# Autodesk Inventor assembly: X_CarriageR_V2_0
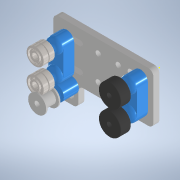
[picture p0: Inventor's stored thumbnail of the model, 180x180]
Saved by Autodesk Inventor 2021 (Build 250183000, 183)
## iProperties
Created: 2021-06-13
Part Number: X_CarriageR_V2_0
Document SubType Name: Assembly
Designer: Jorian Brusind
Author: Jorian Brusind
## Documents named in this file (7)
- C:\Users\Jorian Brusind\Documents\GitHub\PersonalProjects\HyperRail\Inventor Files\X_CarriageR_V2_0.iam
- C:\Users\Jorian Brusind\Documents\GitHub\PersonalProjects\HyperRail\Inventor Files\X_Carriage_Plate.ipt
- C:\Users\Jorian Brusind\Documents\GitHub\PersonalProjects\HyperRail\Inventor Files\11mm_BearingWheel.ipt
- C:\Users\Jorian Brusind\Documents\GitHub\PersonalProjects\HyperRail\Inventor Files\4mm_Roller_Spacer_simple.ipt
- C:\Users\Jorian Brusind\Documents\GitHub\PersonalProjects\HyperRail\Inventor Files\Rollder_Spacer_Single.ipt
- C:\Users\Jorian Brusind\Documents\GitHub\PersonalProjects\HyperRail\Inventor Files\10mm_Idle_Pulley.ipt
- C:\Users\Jorian Brusind\Documents\GitHub\PersonalProjects\HyperRail\Inventor Files\606zz_bearing.ipt
## Components (11 placed, 6 different names)
1. X_Carriage_Plate:1 — Mate:1, Mate:2, Mate:13, Mate:35, Mate:41, Mate:55, Mate:56, Mate:57, Mate:60, Angle:1
2. 11mm_BearingWheel:1 — Mate:1, Flush:2
3. 11mm_BearingWheel:4 — Mate:2, Flush:2, Mate:58
4. 4mm_Roller_Spacer_simple:1 — Mate:13, Mate:50, Mate:53, Mate:54, Mate:59, Mate:60, Angle:1
5. Rollder_Spacer_Single:1 — Mate:35, Mate:40, Mate:41, Mate:42
6. 10mm_Idle_Pulley:1 — Mate:40, Mate:42
7. 606zz_bearing:1 — Mate:48, Mate:49, Mate:59
8. 606zz_bearing:2 — Mate:48, Mate:49, Mate:50
9. 606zz_bearing:3 — Mate:53
10. 606zz_bearing:4 — Mate:54
11. 4mm_Roller_Spacer_simple:2 — Mate:55, Mate:56, Mate:57, Mate:58
## Relationships (22: Mate 20, Flush 1, Angle 1)
- Mate:1: X_Carriage_Plate:1 ↔ 11mm_BearingWheel:1
- Mate:2: X_Carriage_Plate:1 ↔ 11mm_BearingWheel:4
- Flush:2: 11mm_BearingWheel:1 ↔ 11mm_BearingWheel:4
- Mate:13: X_Carriage_Plate:1 ↔ 4mm_Roller_Spacer_simple:1
- Mate:35: X_Carriage_Plate:1 ↔ Rollder_Spacer_Single:1
- Mate:40: Rollder_Spacer_Single:1 ↔ 10mm_Idle_Pulley:1
- Mate:41: X_Carriage_Plate:1 ↔ Rollder_Spacer_Single:1
- Mate:42: Rollder_Spacer_Single:1 ↔ 10mm_Idle_Pulley:1
- Mate:48: 606zz_bearing:1 ↔ 606zz_bearing:2
- Mate:49: 606zz_bearing:1 ↔ 606zz_bearing:2
- Mate:50: 4mm_Roller_Spacer_simple:1 ↔ 606zz_bearing:2
- [Mate]: 606zz_bearing:3 ↔ 606zz_bearing:4
- [Mate]: 606zz_bearing:3 ↔ 606zz_bearing:4
- Mate:53: 4mm_Roller_Spacer_simple:1 ↔ 606zz_bearing:3
- Mate:54: 4mm_Roller_Spacer_simple:1 ↔ 606zz_bearing:4
- Mate:55: X_Carriage_Plate:1 ↔ 4mm_Roller_Spacer_simple:2
- Mate:56: X_Carriage_Plate:1 ↔ 4mm_Roller_Spacer_simple:2
- Mate:57: X_Carriage_Plate:1 ↔ 4mm_Roller_Spacer_simple:2
- Mate:58: 11mm_BearingWheel:4 ↔ 4mm_Roller_Spacer_simple:2
- Mate:59: 4mm_Roller_Spacer_simple:1 ↔ 606zz_bearing:1
- Mate:60 (-15 mm): X_Carriage_Plate:1 ↔ 4mm_Roller_Spacer_simple:1
- Angle:1 (0 deg): X_Carriage_Plate:1 ↔ 4mm_Roller_Spacer_simple:1
## Named parameters: d87_d82 = 0 mm, d88_d83 = 0 mm
